# Autodesk Inventor assembly: Clock sub-assembly
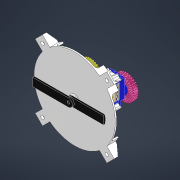
[picture p0: Inventor's stored thumbnail of the model, 180x180]
Saved by Autodesk Inventor 2021 (Build 250183000, 183)
## iProperties
Created: 2021-03-24
Part Number: Clock sub-assembly
Document SubType Name: Assembly
Designer: allen
Author: allen
## Documents named in this file (12)
- C:\Users\Tan Cheong Huat\OneDrive\Stepper motor clock\3D (servo)\Clock sub-assembly.iam
- C:\Users\Tan Cheong Huat\OneDrive\Stepper motor clock\3D (servo)\12T+Gear+Big+Hole.ipt
- C:\Users\Tan Cheong Huat\OneDrive\Stepper motor clock\3D (servo)\32T+Servo+Gear.ipt
- C:\Users\Tan Cheong Huat\OneDrive\Stepper motor clock\3D (servo)\SG90 - Micro Servo 9g - Tower Pro.1.ipt
- C:\Users\Tan Cheong Huat\OneDrive\Stepper motor clock\3D (servo)\Clock body v2.ipt
- C:\Users\Tan Cheong Huat\OneDrive\Stepper motor clock\3D (servo)\Hour shaft test 7.ipt
- C:\Users\Tan Cheong Huat\OneDrive\Stepper motor clock\3D (servo)\Hour hand test 2.ipt
- C:\Users\Tan Cheong Huat\OneDrive\Stepper motor clock\3D (servo)\Minute hand test 2.ipt
- C:\Users\Tan Cheong Huat\OneDrive\Stepper motor clock\3D (servo)\Minute hand shaft.ipt
- C:\Users\Tan Cheong Huat\Documents\Inventor\Content Center Files\R2021\en-US\ISO 7089\ISO 7089 - 3 - 140 HV(1).ipt
- C:\Users\Tan Cheong Huat\OneDrive\Stepper motor clock\3D (servo)\12T+Gear+Small+Hole.ipt
- C:\Users\Tan Cheong Huat\OneDrive\Stepper motor clock\3D (servo)\Hour hand stopper.ipt
## Components (13 placed, 11 different names)
1. 32T+Servo+Gear:1 — Mate:5, Mate:6, Rotation:2
2. Clock body v2:1 — Mate:17, Angle:1, Mate:18, Angle:3, Mate:19, Insert:1, Insert:6
3. SG90 - Micro Servo 9g - Tower Pro.1:1 — Mate:5, Mate:6, Mate:17, Angle:1, Mate:18, Angle:2
4. SG90 - Micro Servo 9g - Tower Pro.1:2 — Mate:8, Mate:9, Angle:2, Angle:3, Mate:19
5. 32T+Servo+Gear:2 — Mate:8, Mate:9, Rotation:1
6. 12T+Gear+Big+Hole:2 — Rotation:1, Insert:7, Rotation:3
7. Hour shaft test 7:1 — Insert:1, Mate:20, Flush:1, Insert:5, Insert:7
8. Hour hand test 2:1 — Mate:20, Flush:1, Insert:3, Rotation:4
9. Minute hand test 2:1 — Insert:2, Insert:4, Rotation:3
10. Minute hand shaft:1 — Insert:4
11. ISO 7089 3:1 — Insert:2, Insert:3
12. 12T+Gear+Small+Hole:1 — Insert:5, Rotation:2, Rotation:4
13. Hour hand stopper:1 — Insert:6
## Relationships (23: Mate 8, Insert 7, RelateRotation 4, Angle 3, Flush 1)
- Mate:5: 32T+Servo+Gear:1 ↔ SG90 - Micro Servo 9g - Tower Pro.1:1
- Mate:6: 32T+Servo+Gear:1 ↔ SG90 - Micro Servo 9g - Tower Pro.1:1
- Mate:8: SG90 - Micro Servo 9g - Tower Pro.1:2 ↔ 32T+Servo+Gear:2
- Mate:9: SG90 - Micro Servo 9g - Tower Pro.1:2 ↔ 32T+Servo+Gear:2
- Rotation:1 [RelateRotation] (1 ul): 32T+Servo+Gear:2 ↔ 12T+Gear+Big+Hole:2
- Mate:17: Clock body v2:1 ↔ SG90 - Micro Servo 9g - Tower Pro.1:1
- Angle:1 (0 deg): Clock body v2:1 ↔ SG90 - Micro Servo 9g - Tower Pro.1:1
- Mate:18: Clock body v2:1 ↔ SG90 - Micro Servo 9g - Tower Pro.1:1
- Angle:2 (0 deg): SG90 - Micro Servo 9g - Tower Pro.1:1 ↔ SG90 - Micro Servo 9g - Tower Pro.1:2
- Angle:3 (0 deg): Clock body v2:1 ↔ SG90 - Micro Servo 9g - Tower Pro.1:2
- Mate:19: Clock body v2:1 ↔ SG90 - Micro Servo 9g - Tower Pro.1:2
- Insert:1: Clock body v2:1 ↔ Hour shaft test 7:1
- Mate:20: Hour shaft test 7:1 ↔ Hour hand test 2:1
- Flush:1: Hour shaft test 7:1 ↔ Hour hand test 2:1
- Insert:2: Minute hand test 2:1 ↔ ISO 7089 3:1
- Insert:3: Hour hand test 2:1 ↔ ISO 7089 3:1
- Insert:4: Minute hand test 2:1 ↔ Minute hand shaft:1
- Insert:5 (-0.7 mm): Hour shaft test 7:1 ↔ 12T+Gear+Small+Hole:1
- Insert:6: Clock body v2:1 ↔ Hour hand stopper:1
- Insert:7 (0.9 mm): 12T+Gear+Big+Hole:2 ↔ Hour shaft test 7:1
- Rotation:2 [RelateRotation] (1 ul): 32T+Servo+Gear:1 ↔ 12T+Gear+Small+Hole:1
- Rotation:3 [RelateRotation] (1 ul): 12T+Gear+Big+Hole:2 ↔ Minute hand test 2:1
- Rotation:4 [RelateRotation] (1 ul): Hour hand test 2:1 ↔ 12T+Gear+Small+Hole:1
